# Autodesk Inventor assembly: gears
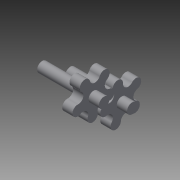
[picture p0: Inventor's stored thumbnail of the model, 180x180]
Saved by Autodesk Inventor 2015 (Build 190159000, 159)
## iProperties
Created: 2015-08-17
Part Number: gears
Document SubType Name: Assembly
Designer: Gustavo
Author: Gustavo
## Documents named in this file (3)
- C:\Users\Gustavo\Desktop\RDECP\stl\gears.iam
- C:\Users\Gustavo\Desktop\RDECP\gearaxle1.ipt
- C:\Users\Gustavo\Desktop\RDECP\gear1.ipt
## Components (4 placed, 2 different names)
1. gearaxle1:1 — Mate:1, Flush:1, Flush:2, Tangent:1
2. gearaxle1:2 — Flush:2, Mate:2, Flush:3, Tangent:1
3. gear1:1 — Mate:1, Flush:1
4. gear1:2 — Mate:2, Flush:3
## Relationships (6: Flush 3, Mate 2, Tangent 1)
- Mate:1: gearaxle1:1 ↔ gear1:1
- Flush:1 (25.4 mm): gearaxle1:1 ↔ gear1:1
- Flush:2: gearaxle1:1 ↔ gearaxle1:2
- Mate:2: gearaxle1:2 ↔ gear1:2
- Flush:3 (25.4 mm): gearaxle1:2 ↔ gear1:2
- Tangent:1 (58.42 mm): gearaxle1:1 ↔ gearaxle1:2
